# Autodesk Inventor assembly: froggy prig disc aero assm
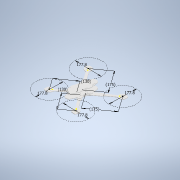
[picture p0: Inventor's stored thumbnail of the model, 180x180]
Saved by Autodesk Inventor 2020 (Build 240168000, 168)
## iProperties
Created: 2022-05-23
Part Number: froggy prig disc aero assm
Document SubType Name: Assembly
Designer: Steven
Author: Steven
## Documents named in this file (5)
- Y:\FPV drone stuff\0 Street League\Frames\experimental-quad-frames\froggy prig disc aero assm.iam
- Y:\FPV drone stuff\0 Street League\Frames\experimental-quad-frames\399 prig z plate.ipt
- Y:\FPV drone stuff\0 Street League\Frames\experimental-quad-frames\399 prig top plate.ipt
- Y:\FPV drone stuff\0 Street League\Frames\experimental-quad-frames\Kauri arm long disc aero.ipt
- Y:\FPV drone stuff\0 Street League\Frames\experimental-quad-frames\Kauri arm short disc aero.ipt
## Components (7 placed, 4 different names)
1. 399 prig z plate:1 — Mate:11, Mate:12, Mate:16, Mate:22, Mate:23, Mate:24, Mate:25
2. 399 prig z plate:2 — Mate:11, Mate:12, Mate:13, Mate:14, Mate:15, Mate:17, Mate:18, Mate:19, Mate:20, Mate:21, Mate:25
3. 399 prig top plate:1 — Mate:13, Mate:14, Mate:15
4. Kauri arm long disc aero:1 — Flush:1, Flush:2, Flush:3, Mate:16, Mate:17, Mate:18
5. Kauri arm long disc aero:2 — Flush:1, Mate:19, Mate:20
6. Kauri arm short disc aero:1 — Flush:2, Mate:21, Mate:22
7. Kauri arm short disc aero:2 — Flush:3, Mate:23, Mate:24
## Relationships (18: Mate 15, Flush 3)
- Mate:11: 399 prig z plate:1 ↔ 399 prig z plate:2
- Mate:12: 399 prig z plate:1 ↔ 399 prig z plate:2
- Mate:13 (25 mm): 399 prig z plate:2 ↔ 399 prig top plate:1
- Mate:14: 399 prig z plate:2 ↔ 399 prig top plate:1
- Mate:15: 399 prig z plate:2 ↔ 399 prig top plate:1
- Flush:1: Kauri arm long disc aero:1 ↔ Kauri arm long disc aero:2
- Flush:2: Kauri arm long disc aero:1 ↔ Kauri arm short disc aero:1
- Flush:3: Kauri arm long disc aero:1 ↔ Kauri arm short disc aero:2
- Mate:16: 399 prig z plate:1 ↔ Kauri arm long disc aero:1
- Mate:17: 399 prig z plate:2 ↔ Kauri arm long disc aero:1
- Mate:18: 399 prig z plate:2 ↔ Kauri arm long disc aero:1
- Mate:19: 399 prig z plate:2 ↔ Kauri arm long disc aero:2
- Mate:20: 399 prig z plate:2 ↔ Kauri arm long disc aero:2
- Mate:21: 399 prig z plate:2 ↔ Kauri arm short disc aero:1
- Mate:22: 399 prig z plate:1 ↔ Kauri arm short disc aero:1
- Mate:23: 399 prig z plate:1 ↔ Kauri arm short disc aero:2
- Mate:24: 399 prig z plate:1 ↔ Kauri arm short disc aero:2
- Mate:25 (6 mm): 399 prig z plate:1 ↔ 399 prig z plate:2
